# Autodesk Inventor assembly: Full overlay hinge for glass door T6
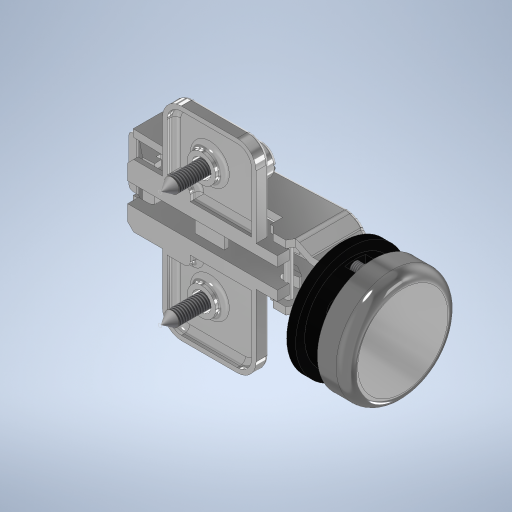
[picture p0: Inventor's stored thumbnail of the model, 512x512]
Saved by Autodesk Inventor 2024 (Build 280153000, 153)
## iProperties
Created: 2014-01-02
Part Number: Full overlay hinge for glass door T6
Document SubType Name: Assembly
Designer: G. Kazokaitis
Author: G. Kazokaitis
## Documents named in this file (23)
- C:\W4INV 2024 Design\LIBRARY\Hinges\HINGE FOR GLASS PANELS.iam
- C:\W4INV 2024 Design\LIBRARY\Hinges\Parts\Hinge for glass panels\Full overlay hinge case.ipt
- C:\W4INV 2024 Design\LIBRARY\Hinges\Parts\Hinge for glass panels\D26 Linkage.ipt
- C:\W4INV 2024 Design\LIBRARY\Hinges\Parts\Hinge for glass panels\D26 Linkages.ipt
- C:\W4INV 2024 Design\LIBRARY\Hinges\Parts\Hinge for glass panels\Case.ipt
- C:\W4INV 2024 Design\LIBRARY\Hinges\Parts\Hinge for glass panels\Half overlay hinge case.ipt
- C:\W4INV 2024 Design\LIBRARY\Hinges\Parts\Hinge for glass panels\PLD26 Linkage.ipt
- C:\W4INV 2024 Design\LIBRARY\Hinges\Parts\Hinge for glass panels\PLD26 Linkages.ipt
- C:\W4INV 2024 Design\LIBRARY\Hinges\Parts\Hinge for glass panels\Insert hinge case.ipt
- C:\W4INV 2024 Design\LIBRARY\Hinges\Parts\Hinge for glass panels\Case\Cup glass T6.ipt
- C:\W4INV 2024 Design\LIBRARY\Hinges\Parts\Hinge for glass panels\Mounting plate.ipt
- Full overlay hinge for glass door T4.iam
- Full overlay hinge for glass door T5.iam
- Full overlay hinge for glass door T6.iam
- Full overlay hinge for glass door T7.iam
- Half overlay hinge for glass door T4.iam
- Half overlay hinge for glass door T5.iam
- Half overlay hinge for glass door T6.iam
- Half overlay hinge for glass door T7.iam
- Inset hinge for glass door T4.iam
- Inset hinge for glass door T5.iam
- Inset hinge for glass door T6.iam
- Inset hinge for glass door T7.iam
## Components (9 placed, 9 different names)
1. Mounting plate:1 — Mate:1, Mate:2, Mate:3, Mate:4, Flush:1, Mate:5, Flush:2, Flush:3, Mate:13, Flush:4, Flush:5, Mate:21
2. Full overlay hinge case:1 — Mate:4, Flush:1, Mate:5, Mate:6, Mate:7, Mate:8, Mate:9, Full overlay opening angle
3. D26 Linkage:1 — Mate:6, Mate:7, Mate:26, Mate:28
4. D26 Linkages:1 — Mate:8, Mate:9, Mate:27
5. Half overlay hinge case:1 — Flush:2, Flush:3, Mate:13, Mate:14, Mate:15, Mate:16, Mate:17, Half overlay opening angle
6. PLD26 Linkage:1 — Mate:14, Mate:15, Mate:22, Mate:25, Mate:29, Mate:31
7. PLD26 Linkages:1 — Mate:16, Mate:17, Mate:23, Mate:24, Mate:30
8. Insert hinge case:1 — Flush:4, Flush:5, Mate:21, Mate:22, Mate:23, Mate:24, Mate:25, Inset opening angle
9. Cup glass T6:1 — Mate:26, Mate:27, Mate:28, Mate:29, Mate:30, Mate:31, Full overlay opening angle, Half overlay opening angle, Inset opening angle
## Relationships (33: Mate 25, Flush 5, Angle 3)
- Mate:1: Mounting plate:1
- Mate:2: Mounting plate:1
- Mate:3: Mounting plate:1
- Mate:4 (2.7 mm): Mounting plate:1 ↔ Full overlay hinge case:1
- Flush:1: Mounting plate:1 ↔ Full overlay hinge case:1
- Mate:5 (5.47 mm): Mounting plate:1 ↔ Full overlay hinge case:1
- Mate:6: Full overlay hinge case:1 ↔ D26 Linkage:1
- Mate:7: Full overlay hinge case:1 ↔ D26 Linkage:1
- Mate:8: Full overlay hinge case:1 ↔ D26 Linkages:1
- Mate:9 (1.3 mm): Full overlay hinge case:1 ↔ D26 Linkages:1
- Flush:2 (-1.1 mm): Mounting plate:1 ↔ Half overlay hinge case:1
- Flush:3: Mounting plate:1 ↔ Half overlay hinge case:1
- Mate:13 (5.47 mm): Mounting plate:1 ↔ Half overlay hinge case:1
- Mate:14: Half overlay hinge case:1 ↔ PLD26 Linkage:1
- Mate:15: Half overlay hinge case:1 ↔ PLD26 Linkage:1
- Mate:16: Half overlay hinge case:1 ↔ PLD26 Linkages:1
- Mate:17 (1.3 mm): Half overlay hinge case:1 ↔ PLD26 Linkages:1
- Flush:4: Mounting plate:1 ↔ Insert hinge case:1
- Flush:5 (0.56 mm): Mounting plate:1 ↔ Insert hinge case:1
- Mate:21 (0.293 mm): Mounting plate:1 ↔ Insert hinge case:1
- Mate:22: PLD26 Linkage:1 ↔ Insert hinge case:1
- Mate:23: PLD26 Linkages:1 ↔ Insert hinge case:1
- Mate:24 (1.3 mm): PLD26 Linkages:1 ↔ Insert hinge case:1
- Mate:25: PLD26 Linkage:1 ↔ Insert hinge case:1
- Mate:26: D26 Linkage:1 ↔ Cup glass T6:1
- Mate:27: D26 Linkages:1 ↔ Cup glass T6:1
- Mate:28 (0.35 mm): D26 Linkage:1 ↔ Cup glass T6:1
- Mate:29: PLD26 Linkage:1 ↔ Cup glass T6:1
- Mate:30: PLD26 Linkages:1 ↔ Cup glass T6:1
- Mate:31 (0.35 mm): PLD26 Linkage:1 ↔ Cup glass T6:1
- Full overlay opening angle [Angle] (90 deg): Full overlay hinge case:1 ↔ Cup glass T6:1
- Half overlay opening angle [Angle] (270 deg): Half overlay hinge case:1 ↔ Cup glass T6:1
- Inset opening angle [Angle] (0 deg): Insert hinge case:1 ↔ Cup glass T6:1
## Named parameters: Edge_distance = 37 mm
